# Autodesk Inventor assembly: Elbow
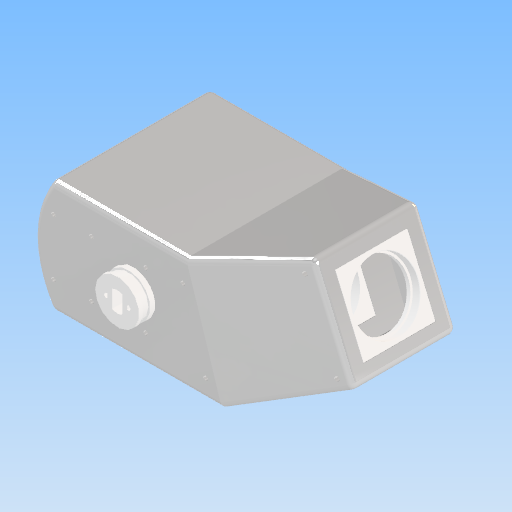
[picture p0: Inventor's stored thumbnail of the model, 512x512]
Saved by Autodesk Inventor 2021 (Build 250183000, 183)
## iProperties
Created: 2020-02-08
Part Number: Elbow
Document SubType Name: Assembly
Designer: JochenAlt
Author: JochenAlt
## Documents named in this file (6)
- D:\Projects\Minibot\CAD\Elbow.iam
- D:\Projects\Minibot\CAD\Elbow.ipt
- D:\Projects\Minibot\CAD\extern\Herkulex\Herkulex DRS-020x.ipt
- D:\Projects\Minibot\CAD\extern\Herkulex\Herkulex DRS-060x.ipt
- C:\Users\Jochen Alt\Documents\Inventor\Content Center Files\R2021\en-US\DIN 912\DIN 912 - M2 x 0.4 x 20 x 19.ipt
- C:\Users\Jochen Alt\Documents\Inventor\Content Center Files\R2021\en-US\DIN 912\DIN 912 - M2 x 0.4 x 8 x 7.ipt
## Components (23 placed, 5 different names)
1. Elbow:1 — Winkel:3, Fluchtend:5, Passend:15, Winkel:4, Passend:17, Insert:1, Insert:4, Insert:5, Insert:6, Insert:7, Insert:8, Insert:9, Insert:10, Insert:11, Insert:12, Insert:13, Insert:14, Insert:15, Insert:16, Insert:17, Insert:18, Insert:19, Insert:20, Insert:21, Insert:22
2. Herkulex DRS-0201:1 — Winkel:4, Passend:17, Passend:18
3. Herkulex DRS-060x:1 — Winkel:3, Fluchtend:5, Passend:15, Passend:18
4. DIN 912 - replaced by DIN EN ISO 4762 M2 x 8:1 — Insert:1
5. DIN 912 - replaced by DIN EN ISO 4762 M2 x 8:2 — Insert:4
6. DIN 912 - replaced by DIN EN ISO 4762 M2 x 8:3 — Insert:5
7. DIN 912 - replaced by DIN EN ISO 4762 M2 x 8:4 — Insert:6
8. DIN 912 - replaced by DIN EN ISO 4762 M2 x 8:5 — Insert:7
9. DIN 912 - replaced by DIN EN ISO 4762 M2 x 8:6 — Insert:8
10. DIN 912 - replaced by DIN EN ISO 4762 M2 x 20:1 — Insert:9
11. DIN 912 - replaced by DIN EN ISO 4762 M2 x 20:2 — Insert:10
12. DIN 912 - replaced by DIN EN ISO 4762 M2 x 20:3 — Insert:11
13. DIN 912 - replaced by DIN EN ISO 4762 M2 x 20:4 — Insert:12
14. DIN 912 - replaced by DIN EN ISO 4762 M2 x 8:7 — Insert:13
15. DIN 912 - replaced by DIN EN ISO 4762 M2 x 8:8 — Insert:14
16. DIN 912 - replaced by DIN EN ISO 4762 M2 x 8:9 — Insert:15
17. DIN 912 - replaced by DIN EN ISO 4762 M2 x 8:10 — Insert:16
18. DIN 912 - replaced by DIN EN ISO 4762 M2 x 8:11 — Insert:17
19. DIN 912 - replaced by DIN EN ISO 4762 M2 x 8:12 — Insert:18
20. DIN 912 - replaced by DIN EN ISO 4762 M2 x 20:5 — Insert:19
21. DIN 912 - replaced by DIN EN ISO 4762 M2 x 20:6 — Insert:20
22. DIN 912 - replaced by DIN EN ISO 4762 M2 x 20:7 — Insert:21
23. DIN 912 - replaced by DIN EN ISO 4762 M2 x 20:8 — Insert:22
## Relationships (26: Insert 20, Mate 3, Angle 2, Flush 1)
- Winkel:3 [Angle] (90 deg): Elbow:1 ↔ Herkulex DRS-060x:1
- Fluchtend:5 [Flush]: Elbow:1 ↔ Herkulex DRS-060x:1
- Passend:15 [Mate]: Elbow:1 ↔ Herkulex DRS-060x:1
- Winkel:4 [Angle] (180 deg): Elbow:1 ↔ Herkulex DRS-0201:1
- Passend:17 [Mate]: Elbow:1 ↔ Herkulex DRS-0201:1
- Passend:18 [Mate] (1.5 mm): Herkulex DRS-0201:1 ↔ Herkulex DRS-060x:1
- Insert:1: Elbow:1 ↔ DIN 912 - replaced by DIN EN ISO 4762 M2 x 8:1
- Insert:4: Elbow:1 ↔ DIN 912 - replaced by DIN EN ISO 4762 M2 x 8:2
- Insert:5: Elbow:1 ↔ DIN 912 - replaced by DIN EN ISO 4762 M2 x 8:3
- Insert:6: Elbow:1 ↔ DIN 912 - replaced by DIN EN ISO 4762 M2 x 8:4
- Insert:7: Elbow:1 ↔ DIN 912 - replaced by DIN EN ISO 4762 M2 x 8:5
- Insert:8: Elbow:1 ↔ DIN 912 - replaced by DIN EN ISO 4762 M2 x 8:6
- Insert:9: Elbow:1 ↔ DIN 912 - replaced by DIN EN ISO 4762 M2 x 20:1
- Insert:10: Elbow:1 ↔ DIN 912 - replaced by DIN EN ISO 4762 M2 x 20:2
- Insert:11: Elbow:1 ↔ DIN 912 - replaced by DIN EN ISO 4762 M2 x 20:3
- Insert:12: Elbow:1 ↔ DIN 912 - replaced by DIN EN ISO 4762 M2 x 20:4
- Insert:13: Elbow:1 ↔ DIN 912 - replaced by DIN EN ISO 4762 M2 x 8:7
- Insert:14: Elbow:1 ↔ DIN 912 - replaced by DIN EN ISO 4762 M2 x 8:8
- Insert:15: Elbow:1 ↔ DIN 912 - replaced by DIN EN ISO 4762 M2 x 8:9
- Insert:16: Elbow:1 ↔ DIN 912 - replaced by DIN EN ISO 4762 M2 x 8:10
- Insert:17: Elbow:1 ↔ DIN 912 - replaced by DIN EN ISO 4762 M2 x 8:11
- Insert:18: Elbow:1 ↔ DIN 912 - replaced by DIN EN ISO 4762 M2 x 8:12
- Insert:19: Elbow:1 ↔ DIN 912 - replaced by DIN EN ISO 4762 M2 x 20:5
- Insert:20: Elbow:1 ↔ DIN 912 - replaced by DIN EN ISO 4762 M2 x 20:6
- Insert:21: Elbow:1 ↔ DIN 912 - replaced by DIN EN ISO 4762 M2 x 20:7
- Insert:22: Elbow:1 ↔ DIN 912 - replaced by DIN EN ISO 4762 M2 x 20:8
